# Autodesk Inventor assembly: vexFrisbeeShooter
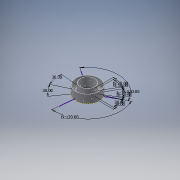
[picture p0: Inventor's stored thumbnail of the model, 180x180]
Saved by Autodesk Inventor 2016 (Build 200138000, 138)
## iProperties
Created: 2015-10-16
Part Number: vexFrisbeeShooter
Document SubType Name: Assembly
Designer: steele
Author: steele
## Documents named in this file (5)
- C:\snobotics\CAD-Development\robSteele\FRC 2013 Ultimate Ascent\vexFrisbeeShooter.iam
- C:\snobotics\CAD-Development\robSteele\FRC 2013 Ultimate Ascent\ShooterBase.ipt
- C:\snobotics\CAD-Development\robSteele\FRC 2013 Ultimate Ascent\vexCam.ipt
- C:\snobotics\CAD-Development\robSteele\FRC 2013 Ultimate Ascent\vexInnerFrisbeeHopper.ipt
- C:\snobotics\CAD-Development\robSteele\FRC 2013 Ultimate Ascent\vexOuterFrisbeeHopper.ipt
## Components (4 placed, 4 different names)
1. ShooterBase:1 — Insert:1, Insert:2, Insert:3
2. vexCam:1 — Insert:1
3. vexInnerFrisbeeHopper:1 — Insert:2
4. vexOuterFrisbeeHopper:1 — Insert:3
## Relationships (3: Insert 3)
- Insert:1 (25.4 mm): ShooterBase:1 ↔ vexCam:1
- Insert:2 (38.1 mm): ShooterBase:1 ↔ vexInnerFrisbeeHopper:1
- Insert:3 (25.4 mm): ShooterBase:1 ↔ vexOuterFrisbeeHopper:1
